# Autodesk Inventor assembly: AM14U3 Long Frame Half
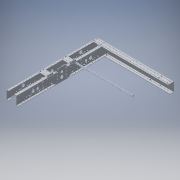
[picture p0: Inventor's stored thumbnail of the model, 180x180]
Saved by Autodesk Inventor 2017 (Build 210142000, 142)
## iProperties
Created: 2018-01-15
Part Number: AM14U3 Long Frame Half
Document SubType Name: Assembly
Designer: S346795925
Author: S346795925
Revision Number: ANY
## Documents named in this file (10)
- \\ad.ocdsb.ca\studenthome\3\S338674153\FRC 2017-18\Robot Mostly Finalized vX\AM14U3 Long Frame Half.iam
- \\ad.ocdsb.ca\studenthome\3\S338674153\FRC 2017-18\Robot Mostly Finalized vX\Churro 3375.ipt
- \\ad.ocdsb.ca\studenthome\3\S338674153\FRC 2017-18\Robot Mostly Finalized vX\FHTS 0.25-20-0.75_FHTS 0.25-20-G-0.75-C.ipt
- \\ad.ocdsb.ca\studenthome\3\S338674153\FRC 2017-18\Robot Mostly Finalized vX\Churro 16250.ipt
- \\ad.ocdsb.ca\studenthome\3\S338674153\FRC 2017-18\Robot Mostly Finalized vX\10-32x0500_shcs_HX-SHCS 0.19-32x1.375x1-C.ipt
- \\ad.ocdsb.ca\studenthome\3\S338674153\FRC 2017-18\Robot Mostly Finalized vX\10-32 Nylock Nut.ipt
- \\ad.ocdsb.ca\studenthome\3\S338674153\FRC 2017-18\Robot Mostly Finalized vX\AM14U3 Inside Sheet Rev2.ipt
- \\ad.ocdsb.ca\studenthome\3\S338674153\FRC 2017-18\Robot Mostly Finalized vX\AM14U3 Outside Sheet Rev1_DefaultSM-FLAT-PATTERN.ipt
- \\ad.ocdsb.ca\studenthome\3\S338674153\FRC 2017-18\Robot Mostly Finalized vX\am-2954 AM14U2 2x3 Hole Bracket.ipt
- \\ad.ocdsb.ca\studenthome\3\S338674153\FRC 2017-18\Robot Mostly Finalized vX\AM14U3 End Sheet Square123.ipt
## Components (60 placed, 60 different names)
1. Churro 3375_80
2. Churro 3375_81
3. Churro 3375_82
4. Churro 3375_83
5. FHTS 0.25-20-0.75_FHTS 0.25-20-G-0.75-C_84
6. FHTS 0.25-20-0.75_FHTS 0.25-20-G-0.75-C_85
7. FHTS 0.25-20-0.75_FHTS 0.25-20-G-0.75-C_86
8. FHTS 0.25-20-0.75_FHTS 0.25-20-G-0.75-C_87
9. FHTS 0.25-20-0.75_FHTS 0.25-20-G-0.75-C_88
10. FHTS 0.25-20-0.75_FHTS 0.25-20-G-0.75-C_89
11. FHTS 0.25-20-0.75_FHTS 0.25-20-G-0.75-C_90
12. FHTS 0.25-20-0.75_FHTS 0.25-20-G-0.75-C_91
13. FHTS 0.25-20-0.75_FHTS 0.25-20-G-0.75-C_92
14. FHTS 0.25-20-0.75_FHTS 0.25-20-G-0.75-C_93
15. Churro 16250_94
16. 10-32x0500_shcs_HX-SHCS 0.19-32x1.375x1-C_95 — Mate:1
17. 10-32x0500_shcs_HX-SHCS 0.19-32x1.375x1-C_96
18. 10-32x0500_shcs_HX-SHCS 0.19-32x1.375x1-C_97 — Mate:2
19. 10-32x0500_shcs_HX-SHCS 0.19-32x1.375x1-C_98
20. 10-32x0500_shcs_HX-SHCS 0.19-32x1.375x1-C_99
21. 10-32x0500_shcs_HX-SHCS 0.19-32x1.375x1-C_100
22. 10-32x0500_shcs_HX-SHCS 0.19-32x1.375x1-C_101
23. 10-32x0500_shcs_HX-SHCS 0.19-32x1.375x1-C_102
24. 10-32x0500_shcs_HX-SHCS 0.19-32x1.375x1-C_103
25. 10-32x0500_shcs_HX-SHCS 0.19-32x1.375x1-C_104
26. 10-32x0500_shcs_HX-SHCS 0.19-32x1.375x1-C_105
27. 10-32x0500_shcs_HX-SHCS 0.19-32x1.375x1-C_106
28. 10-32 Nylock Nut_107
29. 10-32 Nylock Nut_108
30. 10-32 Nylock Nut_109
31. 10-32 Nylock Nut_110
32. 10-32 Nylock Nut_111
33. 10-32 Nylock Nut_112
34. 10-32 Nylock Nut_113
35. 10-32 Nylock Nut_114
36. 10-32 Nylock Nut_115
37. 10-32 Nylock Nut_116
38. 10-32 Nylock Nut_117
39. 10-32 Nylock Nut_118
40. 10-32x0500_shcs_HX-SHCS 0.19-32x1.375x1-C_119
41. 10-32x0500_shcs_HX-SHCS 0.19-32x1.375x1-C_120
42. 10-32x0500_shcs_HX-SHCS 0.19-32x1.375x1-C_121
43. 10-32x0500_shcs_HX-SHCS 0.19-32x1.375x1-C_122
44. 10-32x0500_shcs_HX-SHCS 0.19-32x1.375x1-C_123
45. 10-32x0500_shcs_HX-SHCS 0.19-32x1.375x1-C_124
46. 10-32x0500_shcs_HX-SHCS 0.19-32x1.375x1-C_125
47. 10-32x0500_shcs_HX-SHCS 0.19-32x1.375x1-C_126
48. 10-32 Nylock Nut_127
49. 10-32 Nylock Nut_128
50. 10-32 Nylock Nut_129
51. 10-32 Nylock Nut_130
52. 10-32 Nylock Nut_131
53. 10-32 Nylock Nut_132
54. 10-32 Nylock Nut_133
55. 10-32 Nylock Nut_134
56. AM14U3 Inside Sheet Rev2_136 — Mate:3
57. AM14U3 Outside Sheet Rev1_DefaultSM-FLAT-PATTERN_137
58. am-2954 AM14U2 2x3 Hole Bracket_138
59. am-2954 AM14U2 2x3 Hole Bracket_139
60. AM14U3 End Sheet Square123:3 — Mate:1, Mate:2, Mate:3
## Relationships (3: Mate 3)
- Mate:1: 10-32x0500_shcs_HX-SHCS 0.19-32x1.375x1-C_95 ↔ AM14U3 End Sheet Square123:3
- Mate:2: 10-32x0500_shcs_HX-SHCS 0.19-32x1.375x1-C_97 ↔ AM14U3 End Sheet Square123:3
- Mate:3: AM14U3 Inside Sheet Rev2_136 ↔ AM14U3 End Sheet Square123:3
